# Autodesk Inventor assembly: *New thumb whole v3
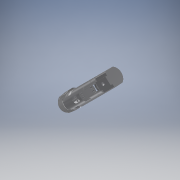
[picture p0: Inventor's stored thumbnail of the model, 180x180]
Saved by Autodesk Inventor 2019 (Build 230136000, 136)
## iProperties
Created: 2019-11-26
Part Number: *New thumb whole v3
Document SubType Name: Assembly
Designer: Administrator
Title: *New thumb whole v3
Author: Administrator
## Documents named in this file (6)
- C:\Users\Bartek\Desktop\reka\fiusion360\Hand show version v5 v4.f3d v1\_New thumb whole v3.iam
- C:\Users\Bartek\Desktop\reka\fiusion360\Hand show version v5 v4.f3d v1\Middle (1) (1).ipt
- C:\Users\Bartek\Desktop\reka\fiusion360\Hand show version v5 v4.f3d v1\Tip (1) (1).ipt
- C:\Users\Bartek\Desktop\reka\fiusion360\Hand show version v5 v4.f3d v1\Lever (4).ipt
- C:\Users\Bartek\Desktop\reka\fiusion360\Hand show version v5 v4.f3d v1\Body (9).ipt
- C:\Users\Bartek\Desktop\reka\fiusion360\Hand show version v5 v4.f3d v1\Base (4).ipt
## Components (5 placed, 5 different names)
1. Middle (1) (1):1 — Zestawiający:3, Zestawiający:4, Zestawiający:7, Zestawiający:9
2. Tip (1) (1):1 — Zestawiający:7, Zestawiający:8, Zestawiający:9
3. Lever (4):1 — Zestawiający:5, Zestawiający:6, Zestawiający:8
4. Body (9):1 — Zestawiający:1, Zestawiający:2
5. Base (4):1 — Zestawiający:1, Zestawiający:2, Zestawiający:3, Zestawiający:4, Zestawiający:5, Zestawiający:6
## Relationships (9: Mate 9)
- Zestawiający:1 [Mate]: Body (9):1 ↔ Base (4):1
- Zestawiający:2 [Mate]: Body (9):1 ↔ Base (4):1
- Zestawiający:3 [Mate]: Middle (1) (1):1 ↔ Base (4):1
- Zestawiający:4 [Mate]: Middle (1) (1):1 ↔ Base (4):1
- Zestawiający:5 [Mate]: Lever (4):1 ↔ Base (4):1
- Zestawiający:6 [Mate]: Lever (4):1 ↔ Base (4):1
- Zestawiający:7 [Mate]: Middle (1) (1):1 ↔ Tip (1) (1):1
- Zestawiający:8 [Mate]: Tip (1) (1):1 ↔ Lever (4):1
- Zestawiający:9 [Mate]: Middle (1) (1):1 ↔ Tip (1) (1):1
